# Autodesk Inventor assembly: Rocker-Bogie-Robot-ASM-01
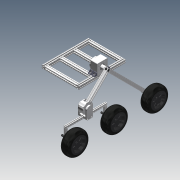
[picture p0: Inventor's stored thumbnail of the model, 180x180]
Saved by Autodesk Inventor 2018.2 (Build 222227000, 227)
## iProperties
Manager: feesmrt
Company: FRANC0R
Created: 2017-12-16
Part Number: Rocker-Bogie-Robot-ASM-01
Material: Generisch
Document SubType Name: Assembly
Designer: feesmrt
Project: Rescue Robot
Cost Center: -
Description: Rocker Bogie Robot Ver 01
Engineer: feesmrt
Authority: feesmrt
Stock Number: Rocker-Bogie-Robot-ASM-01
Author: feesmrt
Title: Rocker Bogie Robot Ver 01
Subject: Rescue Robot
Revision Number: 1
## Documents named in this file (3)
- D:\Programmierung\FRANC0R\CAD\02-Rocker-Bogie-Robot\Rocker-Bogie-Robot-ASM-01.iam
- D:\Programmierung\FRANC0R\CAD\02-Rocker-Bogie-Robot\100-CHASSIS\100-CHASSIS-ASM-01.iam
- D:\Programmierung\FRANC0R\CAD\02-Rocker-Bogie-Robot\200-ROCKER-BOGIE\200-ROCKER-BOGIE-ASM.iam
## Components (2 placed, 2 different names)
1. 100-CHASSIS-ASM-01:1 [sub-assembly] — Fluchtend:1, Fluchtend:2, Passend:1
2. 200-ROCKER-BOGIE-ASM:1 [sub-assembly] — Fluchtend:1, Fluchtend:2, Passend:1
## Relationships (3: Flush 2, Mate 1)
- Fluchtend:1 [Flush]: 100-CHASSIS-ASM-01:1 ↔ 200-ROCKER-BOGIE-ASM:1
- Fluchtend:2 [Flush]: 100-CHASSIS-ASM-01:1 ↔ 200-ROCKER-BOGIE-ASM:1
- Passend:1 [Mate]: 100-CHASSIS-ASM-01:1 ↔ 200-ROCKER-BOGIE-ASM:1
